# Autodesk Inventor assembly: intake
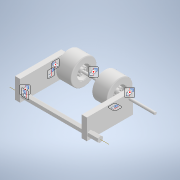
[picture p0: Inventor's stored thumbnail of the model, 180x180]
Saved by Autodesk Inventor 2021 (Build 250183000, 183)
## iProperties
Created: 2020-11-19
Part Number: intake
Document SubType Name: Assembly
Designer: gabe3
Author: gabe3
## Documents named in this file (5)
- D:\robotics\CAD\2020-21-CAD\intake\intake.iam
- D:\robotics\CAD\2020-21-CAD\intake\clolecton wheel holder.ipt
- D:\robotics\CAD\2020-21-CAD\custom parts\.25 axle 9.5in.ipt
- D:\robotics\CAD\COTSParts\Wheels\2.5inFoamWheel250TMD.ipt
- D:\robotics\CAD\2020-21-CAD\custom parts\axles\2in hex 8in.ipt
## Components (7 placed, 4 different names)
1. clolecton wheel holder:1 — Flush:1, Flush:2, Mate:1, Mate:2, Flush:3, Flush:4
2. clolecton wheel holder:2 — Flush:1, Flush:2, Mate:1, Mate:6, Mate:7
3. .25 axle size template:1 — Mate:2, Mate:4, Mate:5, Mate:7, Flush:3
4. 2.5inFoamWheel250TMD:1 — Mate:4
5. 2.5inFoamWheel250TMD:2
6. 2.5inFoamWheel250TMD:3 — Mate:5
7. 2in hex 8in:1 — Mate:6, Flush:4
## Relationships (10: Mate 6, Flush 4)
- Flush:1: clolecton wheel holder:1 ↔ clolecton wheel holder:2
- Flush:2: clolecton wheel holder:1 ↔ clolecton wheel holder:2
- Mate:1 (152.4 mm): clolecton wheel holder:1 ↔ clolecton wheel holder:2
- Mate:2: clolecton wheel holder:1 ↔ .25 axle size template:1
- Mate:4: .25 axle size template:1 ↔ 2.5inFoamWheel250TMD:1
- Mate:5: .25 axle size template:1 ↔ 2.5inFoamWheel250TMD:3
- Mate:6: clolecton wheel holder:2 ↔ 2in hex 8in:1
- Mate:7: clolecton wheel holder:2 ↔ .25 axle size template:1
- Flush:3: clolecton wheel holder:1 ↔ .25 axle size template:1
- Flush:4: clolecton wheel holder:1 ↔ 2in hex 8in:1
